# Autodesk Inventor assembly: ElectronicsBox with components
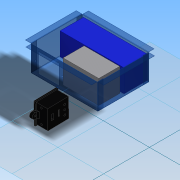
[picture p0: Inventor's stored thumbnail of the model, 180x180]
Saved by Autodesk Inventor 2014 SP2 (Build 180246200, 246)
## iProperties
Created: 2014-06-07
Part Number: ElectronicsBox with components
Document SubType Name: Assembly
Designer: dliu
Author: dliu
## Documents named in this file (6)
- C:\Users\dliu\Dropbox\dbhome\electric-longboard\dliu\Electronics\ElectronicsBox with components.iam
- C:\Users\dliu\Dropbox\dbhome\electric-longboard\dliu\Electronics\ElectronicsBox.ipt
- C:\Users\dliu\Dropbox\dbhome\electric-longboard\dliu\Electronics\Zippy Flightmax 5000 6S 20C.ipt
- C:\Users\dliu\Dropbox\dbhome\electric-longboard\dliu\Electronics\PanelMountNew.ipt
- C:\Users\dliu\Dropbox\dbhome\electric-longboard\dliu\Electronics\ESC HK-200A.ipt
- C:\Users\dliu\Dropbox\dbhome\electric-longboard\dliu\Electronics\HobbyWing EZRUN 150A Pro.ipt
## Components (5 placed, 5 different names)
1. ElectronicsBox:2 — Flush:1, Mate:1, Mate:5, Mate:6
2. Zippy Flightmax 5000 6S 20C:1 — Mate:1
3. PanelMountNew:1 — Mate:6
4. ESC HK-200A:2 — Mate:5
5. HobbyWing EZRUN 150A Pro:1
## Relationships (4: Mate 3, Flush 1)
- Flush:1: ElectronicsBox:2
- Mate:1 (2.54 mm): ElectronicsBox:2 ↔ Zippy Flightmax 5000 6S 20C:1
- Mate:5: ElectronicsBox:2 ↔ ESC HK-200A:2
- Mate:6: ElectronicsBox:2 ↔ PanelMountNew:1
